# Autodesk Inventor assembly: FinalExtruder
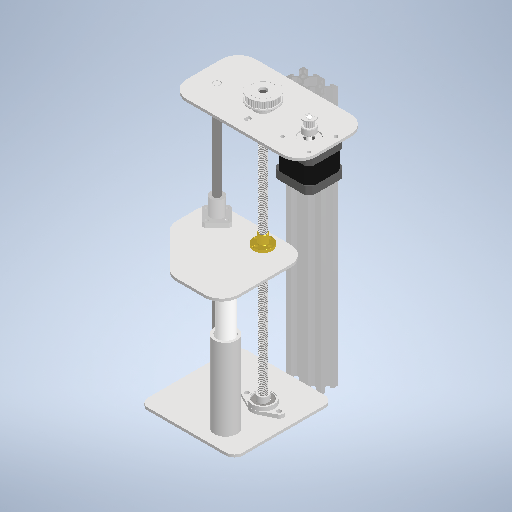
[picture p0: Inventor's stored thumbnail of the model, 512x512]
Saved by Autodesk Inventor 2025.2 (Build 292293000, 293)
## iProperties
Created: 2025-06-23
Part Number: FinalExtruder
Document SubType Name: Assembly
Designer: Simon
Author: Simon
## Documents named in this file (14)
- C:\Users\Simon\Projects\Hydrogel-3D-Printer\Hardware\Bioprinter Machine Design\Extruder Concept 4\SyringeConcept3.iam
- C:\Users\Simon\Projects\Hydrogel-3D-Printer\Hardware\Bioprinter Machine Design\Final System\Final Extruder\Plunger.ipt
- C:\Users\Simon\Projects\Hydrogel-3D-Printer\Hardware\Bioprinter Machine Design\PartsFolder\Stepper_17HS4401.ipt
- C:\Users\Simon\Projects\Hydrogel-3D-Printer\Hardware\Bioprinter Machine Design\PartsFolder\TR8x8-4_Nut.ipt
- C:\Users\Simon\Projects\Hydrogel-3D-Printer\Hardware\Bioprinter Machine Design\PartsFolder\GT2_16T_5.ipt
- C:\Users\Simon\Projects\Hydrogel-3D-Printer\Hardware\Bioprinter Machine Design\PartsFolder\GT2_48T_8.ipt
- C:\Users\Simon\Projects\Hydrogel-3D-Printer\Hardware\Bioprinter Machine Design\PartsFolder\Pillow Block Bearing 1\Zinc Alloy Pillow Block Flange Bearing KFL08 ID-8mm.iam
- C:\Users\Simon\Projects\Hydrogel-3D-Printer\Hardware\Bioprinter Machine Design\Final System\Final Extruder\2040_AluminimProfile_x.ipt
- C:\Users\Simon\Projects\Hydrogel-3D-Printer\Hardware\Bioprinter Machine Design\PartsFolder\LMK8UU.ipt
- C:\Users\Simon\Projects\Hydrogel-3D-Printer\Hardware\Bioprinter Machine Design\Extruder Concept 4\MidPlatform.ipt
- C:\Users\Simon\Projects\Hydrogel-3D-Printer\Hardware\Bioprinter Machine Design\Extruder Concept 4\SyringePlatform.ipt
- C:\Users\Simon\Projects\Hydrogel-3D-Printer\Hardware\Bioprinter Machine Design\Extruder Concept 4\TopPlatform.ipt
- C:\Users\Simon\Projects\Hydrogel-3D-Printer\Hardware\Bioprinter Machine Design\Extruder Concept 4\TR8x8-4_LeadScrew_315.ipt
- C:\Users\Simon\Projects\Hydrogel-3D-Printer\Hardware\Bioprinter Machine Design\Extruder Concept 4\SteelShaft_297.ipt
## Components (14 placed, 13 different names)
1. Stepper_17HS4401:1 — Mate:10, Flush:8, Mate:46, Mate:48, Angle:1
2. TR8x8-4_Nut:2 — Mate:66, Mate:68, Mate:69, Mate:70
3. GT2_16T_5:1 — Mate:10, Flush:8, Flush:9
4. GT2_48T_8:1 — Flush:9, Mate:61
5. Zinc Alloy Pillow Block Flange Bearing KFL08 ID-8mm:1 [sub-assembly] — Mate:53, Mate:54, Mate:55, Mate:60
6. 2040_AluminimProfile_x:1 — Mate:14, Mate:15, Mate:16, Flush:10, Mate:47, Mate:50, Flush:11, Flush:12
7. Plunger:1 — Mate:74, Mate:75
8. Zinc Alloy Pillow Block Flange Bearing KFL08 ID-8mm:2 [sub-assembly] — Mate:56, Mate:57, Mate:58, Mate:62
9. LMK8UU:1 — Mate:65, Mate:71, Mate:72, Mate:73
10. MidPlatform:1 — Mate:67, Mate:68, Mate:69, Mate:70, Mate:71, Mate:72, Mate:73, Mate:75
11. SyringePlatform:1 — Mate:50, Flush:11, Mate:53, Mate:54, Mate:55, Mate:59, Mate:64, Mate:74
12. TopPlatform:1 — Flush:10, Mate:46, Mate:47, Mate:48, Angle:1, Mate:56, Mate:57, Mate:58, Mate:63, Flush:12
13. TR8x8-4_LeadScrew_315:1 — Mate:59, Mate:60, Mate:61, Mate:62, Mate:66
14. SteelShaft_297:1 — Mate:63, Mate:64, Mate:65, Mate:67
## Relationships (37: Mate 31, Flush 5, Angle 1)
- Mate:10: Stepper_17HS4401:1 ↔ GT2_16T_5:1
- Mate:14: 2040_AluminimProfile_x:1
- Mate:15: 2040_AluminimProfile_x:1
- Mate:16: 2040_AluminimProfile_x:1
- Flush:8: Stepper_17HS4401:1 ↔ GT2_16T_5:1
- Flush:9: GT2_16T_5:1 ↔ GT2_48T_8:1
- Flush:10: 2040_AluminimProfile_x:1 ↔ TopPlatform:1
- Mate:46: Stepper_17HS4401:1 ↔ TopPlatform:1
- Mate:47: 2040_AluminimProfile_x:1 ↔ TopPlatform:1
- Mate:48: Stepper_17HS4401:1 ↔ TopPlatform:1
- Angle:1 (0 deg): Stepper_17HS4401:1 ↔ TopPlatform:1
- Mate:50: 2040_AluminimProfile_x:1 ↔ SyringePlatform:1
- Flush:11: 2040_AluminimProfile_x:1 ↔ SyringePlatform:1
- Mate:53: Zinc Alloy Pillow Block Flange Bearing KFL08 ID-8mm:1 ↔ SyringePlatform:1
- Mate:54: Zinc Alloy Pillow Block Flange Bearing KFL08 ID-8mm:1 ↔ SyringePlatform:1
- Mate:55: Zinc Alloy Pillow Block Flange Bearing KFL08 ID-8mm:1 ↔ SyringePlatform:1
- Mate:56: Zinc Alloy Pillow Block Flange Bearing KFL08 ID-8mm:2 ↔ TopPlatform:1
- Mate:57: Zinc Alloy Pillow Block Flange Bearing KFL08 ID-8mm:2 ↔ TopPlatform:1
- Mate:58: Zinc Alloy Pillow Block Flange Bearing KFL08 ID-8mm:2 ↔ TopPlatform:1
- Mate:59: SyringePlatform:1 ↔ TR8x8-4_LeadScrew_315:1
- Mate:60: Zinc Alloy Pillow Block Flange Bearing KFL08 ID-8mm:1 ↔ TR8x8-4_LeadScrew_315:1
- Mate:61: GT2_48T_8:1 ↔ TR8x8-4_LeadScrew_315:1
- Mate:62: Zinc Alloy Pillow Block Flange Bearing KFL08 ID-8mm:2 ↔ TR8x8-4_LeadScrew_315:1
- Mate:63: TopPlatform:1 ↔ SteelShaft_297:1
- Mate:64: SyringePlatform:1 ↔ SteelShaft_297:1
- Mate:65: LMK8UU:1 ↔ SteelShaft_297:1
- Mate:66: TR8x8-4_Nut:2 ↔ TR8x8-4_LeadScrew_315:1
- Mate:67: MidPlatform:1 ↔ SteelShaft_297:1
- Mate:68: TR8x8-4_Nut:2 ↔ MidPlatform:1
- Mate:69: TR8x8-4_Nut:2 ↔ MidPlatform:1
- Mate:70: TR8x8-4_Nut:2 ↔ MidPlatform:1
- Mate:71: LMK8UU:1 ↔ MidPlatform:1
- Mate:72: LMK8UU:1 ↔ MidPlatform:1
- Mate:73: LMK8UU:1 ↔ MidPlatform:1
- Mate:74: Plunger:1 ↔ SyringePlatform:1
- Mate:75: Plunger:1 ↔ MidPlatform:1
- Flush:12: 2040_AluminimProfile_x:1 ↔ TopPlatform:1
